# Autodesk Inventor assembly: Assembly
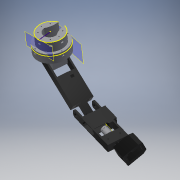
[picture p0: Inventor's stored thumbnail of the model, 180x180]
Saved by Autodesk Inventor 2017 (Build 210142000, 142)
## iProperties
Created: 2017-08-04
Part Number: Assembly
Document SubType Name: Assembly
Designer: Bardo91
Author: Bardo91
## Documents named in this file (9)
- D:\programming\cad_hexacopter\arm_3dog\Assembly.iam
- D:\programming\cad_hexacopter\arm_3dog\Base.ipt
- D:\programming\cad_hexacopter\arm_3dog\rotBase.ipt
- D:\programming\cad_hexacopter\arm_3dog\rotBaseServo.ipt
- D:\programming\cad_hexacopter\arm_3dog\Brazo_p1.ipt
- D:\programming\cad_hexacopter\arm_3dog\Brazo_p2.ipt
- D:\programming\cad_hexacopter\arm_3dog\Brazo_p2_rodamiento1.ipt
- D:\programming\cad_hexacopter\arm_3dog\multiconnectorEndEffector.ipt
- D:\programming\cad_hexacopter\arm_3dog\base_gripper.ipt
## Components (8 placed, 8 different names)
1. Base:1 — Mate:1, Mate:4
2. rotBase:1 — Mate:2, Mate:4, Mate:13
3. rotBaseServo:1 — Mate:1, Mate:2, Mate:5, Mate:13
4. Brazo_p1:1 — Mate:5, Flush:1
5. Brazo_p2:1 — Flush:1, Mate:6, Mate:7, Mate:8
6. Brazo_p2_rodamiento1:1 — Mate:6, Mate:7, Mate:8, Mate:9, Mate:11
7. multiconnectorEndEffector:1 — Mate:9, Mate:10, Mate:11, Mate:12
8. base_gripper:1 — Mate:10, Mate:12
## Relationships (13: Mate 12, Flush 1)
- Mate:1: Base:1 ↔ rotBaseServo:1
- Mate:2: rotBase:1 ↔ rotBaseServo:1
- Mate:4: Base:1 ↔ rotBase:1
- Mate:5: rotBaseServo:1 ↔ Brazo_p1:1
- Flush:1: Brazo_p1:1 ↔ Brazo_p2:1
- Mate:6: Brazo_p2:1 ↔ Brazo_p2_rodamiento1:1
- Mate:7: Brazo_p2:1 ↔ Brazo_p2_rodamiento1:1
- Mate:8: Brazo_p2:1 ↔ Brazo_p2_rodamiento1:1
- Mate:9 (3 mm): Brazo_p2_rodamiento1:1 ↔ multiconnectorEndEffector:1
- Mate:10: multiconnectorEndEffector:1 ↔ base_gripper:1
- Mate:11: Brazo_p2_rodamiento1:1 ↔ multiconnectorEndEffector:1
- Mate:12: multiconnectorEndEffector:1 ↔ base_gripper:1
- Mate:13: rotBase:1 ↔ rotBaseServo:1
